# Autodesk Inventor assembly: hip
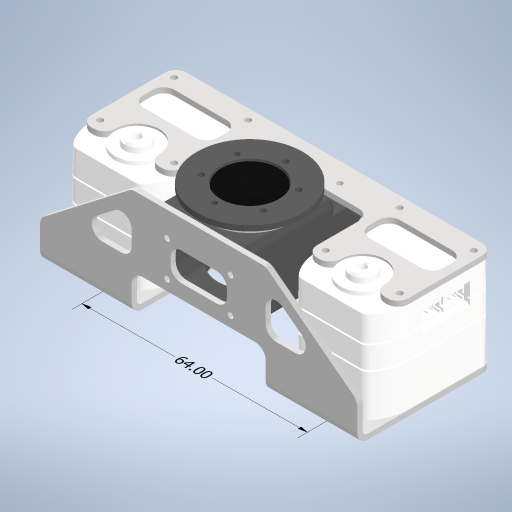
[picture p0: Inventor's stored thumbnail of the model, 512x512]
Saved by Autodesk Inventor 2024.1 (Build 281209000, 209)
## iProperties
Created: 2024-02-12
Part Number: hip
Document SubType Name: Assembly
Designer: hibik
Author: hibik
## Documents named in this file (8)
- C:\Users\hibik\Documents\Robomech\HR\Eglantyne\hard\under_body\hipjoint.iam
- C:\Users\hibik\Documents\Robomech\HR\Eglantyne\hard\needed_model\KRS3300サーボホーン.ipt
- C:\Users\hibik\Documents\Robomech\HR\Eglantyne\hard\under_body\hipjoint_middle.ipt
- C:\Users\hibik\Documents\Robomech\HR\Eglantyne\hard\upper_body\sholder_joint_c.ipt
- C:\Users\hibik\Documents\Robomech\HR\Eglantyne\hard\upper_body\sholder_joint_s.ipt
- C:\Users\hibik\Documents\Robomech\HR\Eglantyne\hard\under_body\hipjoint_front.ipt
- C:\Users\hibik\Documents\Robomech\HR\Eglantyne\hard\under_body\hipjoint_upper.ipt
- C:\Users\hibik\Documents\Robomech\HR\Eglantyne\hard\needed_model\KRS3300モータ.ipt
## Components (10 placed, 7 different names)
1. KRS3300サーボホーン:9 — 挿入:17, 挿入:18, 挿入:19
2. sholder_joint_c:1 — 挿入:19, 挿入:20
3. sholder_joint_s:1 — 挿入:17, 挿入:18, 挿入:20, 挿入:21, 挿入:22
4. hipjoint_middle:1 — 挿入:21, 挿入:22, メイト:1, フラッシュ:1, フラッシュ:2
5. hipjoint_front:1 — メイト:1, フラッシュ:1, フラッシュ:2, 挿入:23, 挿入:24, 角度:1, 角度:2, フラッシュ:3, フラッシュ:4
6. hipjoint_upper:1 — メイト:2, フラッシュ:3, フラッシュ:4
7. KRS3300モータ:1 — 挿入:23, 角度:2, 挿入:25
8. KRS3300モータ:2 — 挿入:24, 角度:1, メイト:2, 挿入:26
9. KRS3300サーボホーン:10 — 挿入:26
10. KRS3300サーボホーン:11 — 挿入:25
## Relationships (18: Insert 10, Flush 4, Mate 2, Angle 2)
- 挿入:17 [Insert]: KRS3300サーボホーン:9 ↔ sholder_joint_s:1
- 挿入:18 [Insert]: KRS3300サーボホーン:9 ↔ sholder_joint_s:1
- 挿入:19 [Insert]: KRS3300サーボホーン:9 ↔ sholder_joint_c:1
- 挿入:20 [Insert]: sholder_joint_c:1 ↔ sholder_joint_s:1
- 挿入:21 [Insert]: sholder_joint_s:1 ↔ hipjoint_middle:1
- 挿入:22 [Insert]: sholder_joint_s:1 ↔ hipjoint_middle:1
- メイト:1 [Mate]: hipjoint_middle:1 ↔ hipjoint_front:1
- フラッシュ:1 [Flush]: hipjoint_middle:1 ↔ hipjoint_front:1
- フラッシュ:2 [Flush] (32.5 mm): hipjoint_middle:1 ↔ hipjoint_front:1
- 挿入:23 [Insert]: hipjoint_front:1 ↔ KRS3300モータ:1
- 挿入:24 [Insert]: hipjoint_front:1 ↔ KRS3300モータ:2
- 角度:1 [Angle] (0 deg): hipjoint_front:1 ↔ KRS3300モータ:2
- 角度:2 [Angle] (0 deg): hipjoint_front:1 ↔ KRS3300モータ:1
- メイト:2 [Mate]: hipjoint_upper:1 ↔ KRS3300モータ:2
- フラッシュ:3 [Flush]: hipjoint_front:1 ↔ hipjoint_upper:1
- フラッシュ:4 [Flush]: hipjoint_front:1 ↔ hipjoint_upper:1
- 挿入:25 [Insert]: KRS3300モータ:1 ↔ KRS3300サーボホーン:11
- 挿入:26 [Insert]: KRS3300モータ:2 ↔ KRS3300サーボホーン:10
